# Autodesk Inventor assembly: center_4p_female
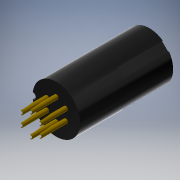
[picture p0: Inventor's stored thumbnail of the model, 180x180]
Saved by Autodesk Inventor 2018 (Build 220112000, 112)
## iProperties
Created: 2019-04-17
Part Number: center_4p_female
Document SubType Name: Assembly
Designer: ZEUSLAP
Author: ZEUSLAP
## Documents named in this file (3)
- C:\Users\Vadim\Desktop\sp16-waterproof-connector-1.snapshot.3\parts\center_6p_female.iam
- C:\Users\Vadim\Desktop\sp16-waterproof-connector-1.snapshot.3\parts\pin_1mm.ipt
- C:\Users\Vadim\Desktop\sp16-waterproof-connector-1.snapshot.3\parts\center_6p_female_body.ipt
## Components (7 placed, 2 different names)
1. center_6p_female_body:1 — Angle:1, Angle:2, Angle:3, Angle:4, Mate:5, Angle:5, Angle:6, Angle:7, Angle:8, Angle:9, Flush:4, Mate:11, Mate:12, Mate:13, Mate:14, Mate:15, Angle:10, Angle:11, Mate:16
2. pin_1mm:1 — Angle:2, Flush:1, Flush:2, Angle:9, Mate:14
3. pin_1mm:2 — Angle:3, Flush:2, Flush:3, Angle:8, Mate:15
4. pin_1mm:3 — Angle:4, Flush:3, Angle:7, Flush:5, Mate:13, Flush:6
5. pin_1mm:4 — Angle:1, Flush:1, Angle:6, Flush:4, Mate:12
6. pin_1mm:5 — Flush:5, Mate:11
7. pin_1mm:6 — Angle:10, Angle:11, Mate:16, Flush:6
## Relationships (24: Angle 11, Mate 7, Flush 6)
- Angle:1 (180 deg): center_6p_female_body:1 ↔ pin_1mm:4
- Angle:2 (180 deg): center_6p_female_body:1 ↔ pin_1mm:1
- Angle:3 (180 deg): center_6p_female_body:1 ↔ pin_1mm:2
- Angle:4 (180 deg): center_6p_female_body:1 ↔ pin_1mm:3
- Flush:1: pin_1mm:1 ↔ pin_1mm:4
- Flush:2: pin_1mm:1 ↔ pin_1mm:2
- Flush:3: pin_1mm:2 ↔ pin_1mm:3
- Mate:5: center_6p_female_body:1
- Angle:5 (180 deg): center_6p_female_body:1
- Angle:6 (90 deg): center_6p_female_body:1 ↔ pin_1mm:4
- Angle:7 (270 deg): center_6p_female_body:1 ↔ pin_1mm:3
- Angle:8 (270 deg): center_6p_female_body:1 ↔ pin_1mm:2
- Angle:9 (270 deg): center_6p_female_body:1 ↔ pin_1mm:1
- Flush:4 (6 mm): center_6p_female_body:1 ↔ pin_1mm:4
- Flush:5: pin_1mm:3 ↔ pin_1mm:5
- Mate:11: center_6p_female_body:1 ↔ pin_1mm:5
- Mate:12: center_6p_female_body:1 ↔ pin_1mm:4
- Mate:13: center_6p_female_body:1 ↔ pin_1mm:3
- Mate:14: center_6p_female_body:1 ↔ pin_1mm:1
- Mate:15: center_6p_female_body:1 ↔ pin_1mm:2
- Angle:10 (180 deg): center_6p_female_body:1 ↔ pin_1mm:6
- Angle:11 (90 deg): center_6p_female_body:1 ↔ pin_1mm:6
- Mate:16: center_6p_female_body:1 ↔ pin_1mm:6
- Flush:6: pin_1mm:3 ↔ pin_1mm:6
